# Autodesk Inventor assembly: złożenie pedały
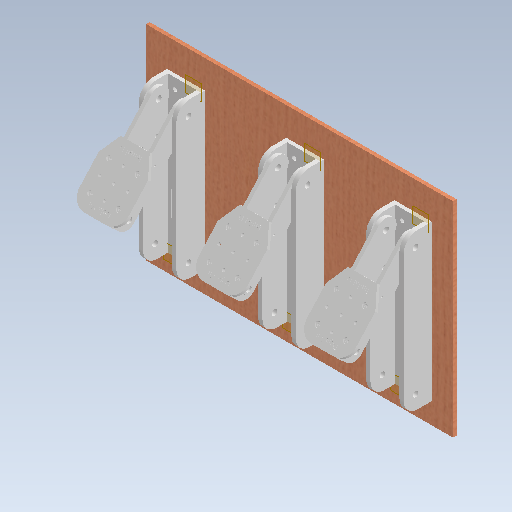
[picture p0: Inventor's stored thumbnail of the model, 512x512]
Saved by Autodesk Inventor 2021 (Build 250183000, 183)
## iProperties
Created: 2022-04-14
Part Number: złożenie pedały
Document SubType Name: Assembly
Designer: Łukasz
Author: Łukasz
## Documents named in this file (3)
- E:\Pliki inventor i stl\motion platform\złożenie pedały.iam
- E:\Pliki inventor i stl\motion platform\podstawa pod gaz.ipt
- E:\Pliki inventor i stl\motion platform\złożenie gaz.iam
## Components (4 placed, 2 different names)
1. podstawa pod gaz:1 — Mate:1, Flush:1, Flush:2, Mate:2, Flush:3, Flush:4, Mate:3, Flush:5
2. złożenie gaz:1 [sub-assembly] — Mate:1, Flush:1, Flush:2
3. złożenie gaz:2 [sub-assembly] — Mate:2, Flush:3, Flush:4, Mate:4
4. złożenie gaz:3 [sub-assembly] — Mate:3, Flush:5, Mate:4
## Relationships (9: Flush 5, Mate 4)
- Mate:1: podstawa pod gaz:1 ↔ złożenie gaz:1
- Flush:1 (30 mm): podstawa pod gaz:1 ↔ złożenie gaz:1
- Flush:2 (30 mm): podstawa pod gaz:1 ↔ złożenie gaz:1
- Mate:2: podstawa pod gaz:1 ↔ złożenie gaz:2
- Flush:3 (30 mm): podstawa pod gaz:1 ↔ złożenie gaz:2
- Flush:4 (30 mm): podstawa pod gaz:1 ↔ złożenie gaz:2
- Mate:3: podstawa pod gaz:1 ↔ złożenie gaz:3
- Flush:5 (30 mm): podstawa pod gaz:1 ↔ złożenie gaz:3
- Mate:4 (100 mm): złożenie gaz:2 ↔ złożenie gaz:3
